# Autodesk Inventor assembly: Assembly_assignment
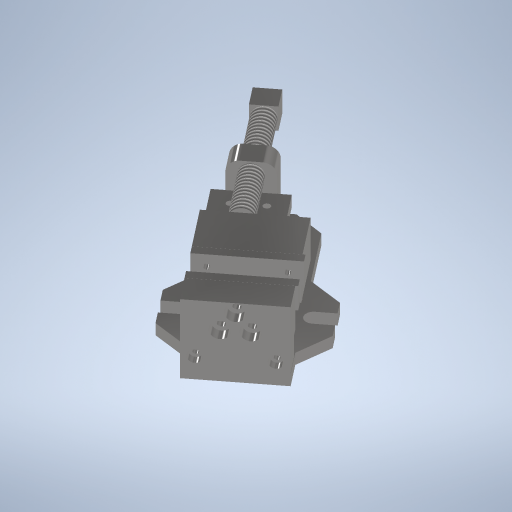
[picture p0: Inventor's stored thumbnail of the model, 512x512]
Saved by Autodesk Inventor 2023.2 (Build 272271000, 271)
## iProperties
Created: 2023-02-07
Part Number: Assembly_assignment
Document SubType Name: Assembly
Designer: Ayush
Author: Ayush
## Documents named in this file (9)
- F:\MS\SRH study\CAD projects\Class4\3114516_Machine_vice\Assembly_assignment.iam
- F:\MS\SRH study\CAD projects\Class4\3114516_Machine_vice\Grundplatte.ipt
- F:\MS\SRH study\CAD projects\Class4\3114516_Machine_vice\Feste Backe.ipt
- F:\MS\SRH study\CAD projects\Class4\3114516_Machine_vice\Fuhrung.ipt
- F:\MS\SRH study\CAD projects\Class4\3114516_Machine_vice\spindel sockel.ipt
- F:\MS\SRH study\CAD projects\Class4\3114516_Machine_vice\Spannbacke.ipt
- F:\MS\SRH study\CAD projects\Class4\3114516_Machine_vice\Lose backe.ipt
- F:\MS\SRH study\CAD projects\Class4\3114516_Machine_vice\Trapezspindle.ipt
- F:\MS\SRH study\CAD projects\Class4\3114516_Machine_vice\Bolt.ipt
## Components (10 placed, 9 different names)
1. Grundplatte:2 — Mate:1, Flush:1, Mate:2, Mate:9, Mate:12
2. Feste Backe:1 — Mate:1, Flush:1, Mate:2, Mate:7, Mate:8, Flush:2, Flush:3, Mate:10, Flush:6
3. spindel sockel:1 — Mate:11, Flush:4, Mate:12, Mate:16
4. Spannbacke:1 — Mate:7, Mate:8, Flush:2, Flush:6
5. Fuhrung:1 — Mate:9, Flush:3, Mate:10, Mate:11, Flush:4, Mate:13, Flush:5
6. Lose backe:1 — Mate:13, Flush:5, Mate:14, Mate:15, Flush:7, Mate:17, Mate:18
7. Spannbacke:3 — Mate:14, Mate:15, Flush:7
8. Trapezspindle:1 — Mate:16
9. Fuhrung1 — Mate:17
10. Fuhrungs — Mate:18
## Relationships (21: Mate 14, Flush 7)
- Mate:1: Grundplatte:2 ↔ Feste Backe:1
- Flush:1: Grundplatte:2 ↔ Feste Backe:1
- Mate:2: Grundplatte:2 ↔ Feste Backe:1
- Mate:7: Feste Backe:1 ↔ Spannbacke:1
- Mate:8: Feste Backe:1 ↔ Spannbacke:1
- Flush:2: Feste Backe:1 ↔ Spannbacke:1
- Mate:9: Grundplatte:2 ↔ Fuhrung:1
- Flush:3: Feste Backe:1 ↔ Fuhrung:1
- Mate:10: Feste Backe:1 ↔ Fuhrung:1
- Mate:11: spindel sockel:1 ↔ Fuhrung:1
- Flush:4: spindel sockel:1 ↔ Fuhrung:1
- Mate:12: Grundplatte:2 ↔ spindel sockel:1
- Mate:13: Fuhrung:1 ↔ Lose backe:1
- Flush:5: Fuhrung:1 ↔ Lose backe:1
- Mate:14: Lose backe:1 ↔ Spannbacke:3
- Mate:15: Lose backe:1 ↔ Spannbacke:3
- Flush:6: Feste Backe:1 ↔ Spannbacke:1
- Flush:7: Lose backe:1 ↔ Spannbacke:3
- Mate:16: spindel sockel:1 ↔ Trapezspindle:1
- Mate:17: Lose backe:1 ↔ Fuhrung1
- Mate:18: Lose backe:1 ↔ Fuhrungs
